# Autodesk Inventor assembly: Assembly_Cube_Lens_holder_25mm_v3
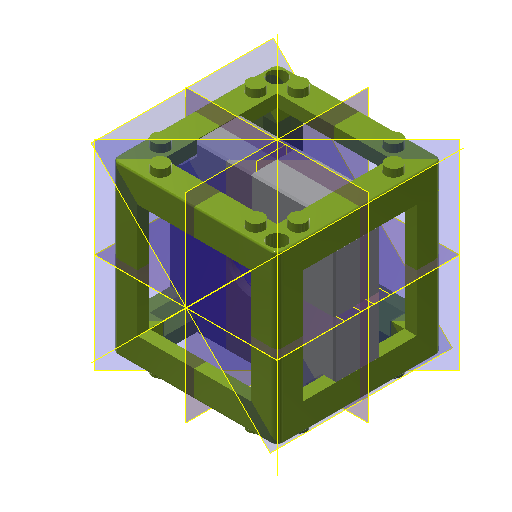
[picture p0: Inventor's stored thumbnail of the model, 512x512]
Saved by Autodesk Inventor 2022 (Build 260153000, 153)
## iProperties
Created: 2020-11-11
Part Number: Assembly_Cube_Lens_holder_25mm_v3
Document SubType Name: Assembly
Designer: marsikovabarbora
Author: marsikovabarbora
## Documents named in this file (5)
- C:\Users\diederichbenedict\Dropbox\Dokumente\Promotion\PROJECTS\openUC2-CAD\INVENTOR\Assembly_Cube_Lens_holder_25mm_v3.iam
- C:\Users\diederichbenedict\Dropbox\Dokumente\Promotion\PROJECTS\openUC2-CAD\INVENTOR\Assembly_Cube_empty_IM_v3.iam
- C:\Users\diederichbenedict\Dropbox\Dokumente\Promotion\PROJECTS\openUC2-CAD\INVENTOR\00_Lens_neg_50mm_India.ipt
- C:\Users\diederichbenedict\Dropbox\Dokumente\Promotion\PROJECTS\openUC2-CAD\INVENTOR\20_Cube_Insert_Lens_neg_Diameter_15mm_generic_Lid.ipt
- C:\Users\diederichbenedict\Dropbox\Dokumente\Promotion\PROJECTS\openUC2-CAD\INVENTOR\20_Cube_Insert_Lens_neg_Diameter_15mm_generic.ipt
## Components (4 placed, 4 different names)
1. Assembly_Cube_empty_IM_v3:1 [sub-assembly] — Mate:1, Mate:2, Mate:3, Passend:9, Passend:10
2. 20_Cube_Insert_Lens_neg_Diameter_15mm_generic:1 — Passend:9, Passend:10, Einfügen:1, Einfügen:2
3. 00_Lens_neg_50mm_India:1 — Einfügen:1
4. 20_Cube_Insert_Lens_neg_Diameter_15mm_generic_Lid:1 — Einfügen:2
## Relationships (7: Mate 5, Insert 2)
- Mate:1: Assembly_Cube_empty_IM_v3:1
- Mate:2: Assembly_Cube_empty_IM_v3:1
- Mate:3: Assembly_Cube_empty_IM_v3:1
- Passend:9 [Mate]: Assembly_Cube_empty_IM_v3:1 ↔ 20_Cube_Insert_Lens_neg_Diameter_15mm_generic:1
- Passend:10 [Mate]: Assembly_Cube_empty_IM_v3:1 ↔ 20_Cube_Insert_Lens_neg_Diameter_15mm_generic:1
- Einfügen:1 [Insert]: 20_Cube_Insert_Lens_neg_Diameter_15mm_generic:1 ↔ 00_Lens_neg_50mm_India:1
- Einfügen:2 [Insert]: 20_Cube_Insert_Lens_neg_Diameter_15mm_generic:1 ↔ 20_Cube_Insert_Lens_neg_Diameter_15mm_generic_Lid:1
